# Autodesk Inventor assembly: 001_pakutta_L
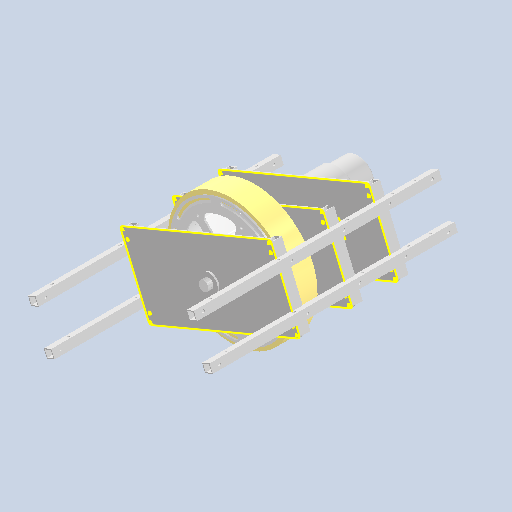
[picture p0: Inventor's stored thumbnail of the model, 512x512]
Saved by Autodesk Inventor 2025.1 (Build 291241000, 241)
## iProperties
Created: 2024-10-03
Part Number: 001_pakutta_L
Document SubType Name: Assembly
Designer: yuki0520
Author: yuki0520
## Documents named in this file (12)
- C:\Users\yuki0520\OneDrive\ドキュメント\Inventor\2025_nhk\tanaka\nageru\pakuriz\001_pakutta_L.iam
- C:\Users\yuki0520\OneDrive\ドキュメント\Inventor\2025_nhk\tanaka\nageru\pakuriz\tire.iam
- C:\Users\yuki0520\OneDrive\ドキュメント\Inventor\2025_nhk\tanaka\nageru\pakuriz\TH22_Bar_roller_sn.ipt
- C:\Users\yuki0520\OneDrive\ドキュメント\Inventor\2025_nhk\tanaka\nageru\inventorパーツリスト\モーター\775\RS-775GM.ipt
- C:\Users\yuki0520\OneDrive\ドキュメント\Inventor\2025_nhk\tanaka\nageru\inventorパーツリスト\モーター\775\RS-775GM_004GH_sn.ipt
- C:\Users\yuki0520\OneDrive\ドキュメント\Inventor\2025_nhk\tanaka\nageru\pakuriz\TH22_Bar_motor_roller_sn.ipt
- C:\Users\yuki0520\OneDrive\ドキュメント\Inventor\2025_nhk\tanaka\nageru\pakuriz\canon_plate_motor.ipt
- C:\Users\yuki0520\OneDrive\ドキュメント\Inventor\2025_nhk\tanaka\nageru\pakuriz\canon_plate.ipt
- C:\Users\yuki0520\OneDrive\ドキュメント\Inventor\2025_nhk\tanaka\nageru\pakuriz\kaku_1010_120.ipt
- C:\Users\yuki0520\OneDrive\ドキュメント\Inventor\2025_nhk\tanaka\nageru\pakuriz\kaku_1010_200.ipt
- C:\Users\yuki0520\OneDrive\ドキュメント\Inventor\2025_nhk\tanaka\nageru\pakuriz\gear_kiseihin.iam
- C:\Users\yuki0520\OneDrive\ドキュメント\Inventor\2025_nhk\tanaka\nageru\pakuriz\bear_12_18.ipt
## Components (22 placed, 11 different names)
1. tire:1 [sub-assembly] — メイト:1, メイト:3
2. TH22_Bar_roller_sn:1 — メイト:1, メイト:3, メイト:9, メイト:10, メイト:11, メイト:15, メイト:16, メイト:18
3. RS-775GM:1 — メイト:4, 正接:1
4. RS-775GM_004GH_sn:1 — メイト:4, 正接:1, メイト:5, メイト:7, 挿入:17, 挿入:18
5. TH22_Bar_motor_roller_sn:1 — メイト:5, メイト:7, メイト:8, メイト:12, メイト:13
6. canon_plate_motor:1 — メイト:8, メイト:9, 挿入:1, 挿入:2, 挿入:3, 挿入:4, 挿入:17, 挿入:18, メイト:17
7. canon_plate:1 — メイト:10, 挿入:5, 挿入:6, 挿入:7, 挿入:8, メイト:14, メイト:18
8. kaku_1010_120:1 — 挿入:3, 挿入:4, 挿入:11, 挿入:16
9. kaku_1010_120:2 — 挿入:1, 挿入:2, 挿入:9, 挿入:14
10. kaku_1010_120:3 — 挿入:5, 挿入:6, 挿入:10, 挿入:13
11. kaku_1010_120:4 — 挿入:7, 挿入:8, 挿入:12, 挿入:15
12. kaku_1010_200:1 — 挿入:9, 挿入:10
13. kaku_1010_200:2 — 挿入:11, 挿入:12, 挿入:24
14. kaku_1010_200:3 — 挿入:13, 挿入:14, 挿入:23
15. kaku_1010_200:4 — 挿入:15, 挿入:16
16. gear_kiseihin:1 [sub-assembly] — メイト:11, メイト:12, メイト:13
17. bear_12_18:1 — メイト:14, メイト:15
18. bear_12_18:2 — メイト:16, メイト:17
19. canon_plate_motor:2 — メイト:20
20. kaku_1010_120:5 — 挿入:24
21. kaku_1010_120:6 — 挿入:23
22. bear_12_18:3 — メイト:20
## Relationships (43: Insert 24, Mate 18, Tangent 1)
- メイト:1 [Mate]: tire:1 ↔ TH22_Bar_roller_sn:1
- メイト:3 [Mate]: tire:1 ↔ TH22_Bar_roller_sn:1
- メイト:4 [Mate]: RS-775GM:1 ↔ RS-775GM_004GH_sn:1
- 正接:1 [Tangent]: RS-775GM:1 ↔ RS-775GM_004GH_sn:1
- メイト:5 [Mate]: RS-775GM_004GH_sn:1 ↔ TH22_Bar_motor_roller_sn:1
- メイト:7 [Mate]: RS-775GM_004GH_sn:1 ↔ TH22_Bar_motor_roller_sn:1
- メイト:8 [Mate]: TH22_Bar_motor_roller_sn:1 ↔ canon_plate_motor:1
- メイト:9 [Mate]: TH22_Bar_roller_sn:1 ↔ canon_plate_motor:1
- メイト:10 [Mate]: TH22_Bar_roller_sn:1 ↔ canon_plate:1
- 挿入:1 [Insert]: canon_plate_motor:1 ↔ kaku_1010_120:2
- 挿入:2 [Insert]: canon_plate_motor:1 ↔ kaku_1010_120:2
- 挿入:3 [Insert]: canon_plate_motor:1 ↔ kaku_1010_120:1
- 挿入:4 [Insert]: canon_plate_motor:1 ↔ kaku_1010_120:1
- 挿入:5 [Insert]: canon_plate:1 ↔ kaku_1010_120:3
- 挿入:6 [Insert]: canon_plate:1 ↔ kaku_1010_120:3
- 挿入:7 [Insert]: canon_plate:1 ↔ kaku_1010_120:4
- 挿入:8 [Insert]: canon_plate:1 ↔ kaku_1010_120:4
- 挿入:9 [Insert]: kaku_1010_120:2 ↔ kaku_1010_200:1
- 挿入:10 [Insert]: kaku_1010_120:3 ↔ kaku_1010_200:1
- 挿入:11 [Insert]: kaku_1010_120:1 ↔ kaku_1010_200:2
- 挿入:12 [Insert]: kaku_1010_120:4 ↔ kaku_1010_200:2
- 挿入:13 [Insert]: kaku_1010_120:3 ↔ kaku_1010_200:3
- 挿入:14 [Insert]: kaku_1010_120:2 ↔ kaku_1010_200:3
- 挿入:15 [Insert]: kaku_1010_120:4 ↔ kaku_1010_200:4
- 挿入:16 [Insert]: kaku_1010_120:1 ↔ kaku_1010_200:4
- メイト:11 [Mate]: TH22_Bar_roller_sn:1 ↔ gear_kiseihin:1
- 挿入:17 [Insert]: RS-775GM_004GH_sn:1 ↔ canon_plate_motor:1
- 挿入:18 [Insert]: RS-775GM_004GH_sn:1 ↔ canon_plate_motor:1
- メイト:12 [Mate]: TH22_Bar_motor_roller_sn:1 ↔ gear_kiseihin:1
- メイト:13 [Mate]: TH22_Bar_motor_roller_sn:1 ↔ gear_kiseihin:1
- メイト:14 [Mate]: canon_plate:1 ↔ bear_12_18:1
- メイト:15 [Mate]: TH22_Bar_roller_sn:1 ↔ bear_12_18:1
- メイト:16 [Mate]: TH22_Bar_roller_sn:1 ↔ bear_12_18:2
- メイト:17 [Mate]: canon_plate_motor:1 ↔ bear_12_18:2
- メイト:18 [Mate] (5 mm): TH22_Bar_roller_sn:1 ↔ canon_plate:1
- [Insert]: canon_plate_motor:2 ↔ kaku_1010_120:6
- [Insert]: canon_plate_motor:2 ↔ kaku_1010_120:6
- [Insert]: canon_plate_motor:2 ↔ kaku_1010_120:5
- [Insert]: canon_plate_motor:2 ↔ kaku_1010_120:5
- [Mate]: canon_plate_motor:2 ↔ bear_12_18:3
- メイト:20 [Mate]: canon_plate_motor:2 ↔ bear_12_18:3
- 挿入:23 [Insert]: kaku_1010_200:3 ↔ kaku_1010_120:6
- 挿入:24 [Insert]: kaku_1010_200:2 ↔ kaku_1010_120:5
## Named parameters: d54_d52 = 0 mm, d55_d25 = 0 mm, d56_d26 = 0 mm, d57_d27 = 0 mm, d58_d28 = 0 mm
